# Autodesk Inventor assembly: BLACK SERVO
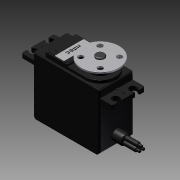
[picture p0: Inventor's stored thumbnail of the model, 180x180]
Saved by Autodesk Inventor 2012 (Build 160160000, 160)
## iProperties
Created: 2010-12-08
Part Number: BLACK SERVO
Document SubType Name: Assembly
Designer: AndrewRemmers
Author: AndrewRemmers
## Documents named in this file (11)
- C:\Users\Andrew\Documents\Inventor\FTC 2010 GET OVER IT\FTC CAD Database\FTC CAD Files\Servos\BLACK SERVO.iam
- C:\Users\Andrew\Documents\Inventor\FTC 2010 GET OVER IT\Imported Components\180 Degree Servo\Part2.ipt
- C:\Users\Andrew\Documents\Inventor\FTC 2010 GET OVER IT\Imported Components\180 Degree Servo\Part4.ipt
- C:\Users\Andrew\Documents\Inventor\FTC 2010 GET OVER IT\Imported Components\180 Degree Servo\Part6.ipt
- C:\Users\Andrew\Documents\Inventor\FTC 2010 GET OVER IT\Imported Components\180 Degree Servo\Part8.ipt
- C:\Users\Andrew\Documents\Inventor\FTC 2010 GET OVER IT\Imported Components\180 Degree Servo\Part10.ipt
- C:\Users\Andrew\Documents\Inventor\FTC 2010 GET OVER IT\Imported Components\180 Degree Servo\Part12.ipt
- C:\Users\Andrew\Documents\Inventor\FTC 2010 GET OVER IT\Imported Components\180 Degree Servo\Part14.ipt
- C:\Users\Andrew\Documents\Inventor\FTC 2010 GET OVER IT\Imported Components\180 Degree Servo\Part16.ipt
- C:\Users\Andrew\Documents\Inventor\FTC 2010 GET OVER IT\Imported Components\180 Degree Servo\Part18.ipt
- C:\Users\Andrew\Documents\Inventor\FTC 2010 GET OVER IT\Imported Components\180 Degree Servo\Part20.ipt
## Components (10 placed, 10 different names)
1. Part2:1 — Insert:1, Insert:2
2. Part4:1 — Insert:2
3. Part6:1
4. Part8:1
5. Part10:1
6. Part12:1
7. Part14:1
8. Part16:1
9. Part18:1
10. Part20:1 — Insert:1
## Relationships (2: Insert 2)
- Insert:1: Part2:1 ↔ Part20:1
- Insert:2: Part2:1 ↔ Part4:1
